# Autodesk Inventor assembly: Sub sytem 3 (2)
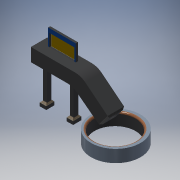
[picture p0: Inventor's stored thumbnail of the model, 180x180]
Saved by Autodesk Inventor 2019 (Build 230136000, 136)
## iProperties
Created: 2020-05-13
Part Number: Sub sytem 3 (2)
Document SubType Name: Assembly
Designer: Adityan Matthew
Author: Adityan Matthew
## Documents named in this file (3)
- D:\Sub sytem 3 (2).iam
- D:\k.ipt
- D:\k2.ipt
## Components (3 placed, 2 different names)
1. k:1 — Mate:1, Mate:2, Mate:3, Mate:4
2. k2:1 — Mate:2, Mate:3, Mate:4
3. k2:2 — Mate:1
## Relationships (4: Mate 4)
- Mate:1: k:1 ↔ k2:2
- Mate:2: k:1 ↔ k2:1
- Mate:3: k:1 ↔ k2:1
- Mate:4: k:1 ↔ k2:1
